# Autodesk Inventor assembly: 90 degree curved shooter v1
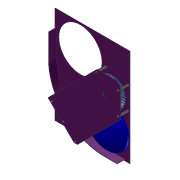
[picture p0: Inventor's stored thumbnail of the model, 180x180]
Saved by Autodesk Inventor 2012 (Build 160160000, 160)
## iProperties
Created: 2013-01-15
Part Number: 90 degree curved shooter v1
Document SubType Name: Assembly
Designer: William
Mass: 2029.94 g
Surface Area: 13536.5 cm^2
Volume: 1773.91 cm^3
Density: 1.14433 g/cm^3
Author: William
## Documents named in this file (10)
- Z:\UserData\Documents\Inventor\team1885frc\Robot2013\Launcher\90 degree curved shooter v1.iam
- Z:\UserData\Documents\Inventor\team1885frc\Robot2013\Launcher\Shooter Plate.ipt
- Z:\UserData\Documents\Inventor\team1885frc\Robot2013\Launcher\Shooter Curve.ipt
- Z:\UserData\Documents\Inventor\team1885frc\Hardware\Bearings\500id_1.125od_closed_flange_bearing.ipt
- Z:\UserData\Documents\Inventor\team1885frc\Robot2013\Game\disc.ipt
- Z:\UserData\Documents\Inventor\team1885frc\Robot2013\Launcher\Shooter Plate top.ipt
- Z:\UserData\Documents\Inventor\team1885frc\AndyMark\PneumaticWheel_am-0970\PneumaticWheel_am-0970.iam
- Z:\UserData\Documents\Inventor\team1885frc\VEXPro\VersaHub\217-2592.20121203.ipt
- Z:\UserData\Documents\Inventor\team1885frc\Robot2013\LauncherRearrange\UpperPlateStandoff.ipt
- Z:\UserData\Documents\Inventor\team1885frc\Hardware\Bolts\Bolt_0.25_20_0.75len_SocketHead.ipt
## Components (26 placed, 9 different names)
1. Shooter Plate:1 — Flush:1, Flush:2, Mate:3, Mate:16, Mate:100, Mate:101, Mate:121, Mate:122, Mate:123, Mate:124, Mate:125, Mate:126, Mate:136, Mate:137, Mate:138, Mate:139, Mate:140, Mate:141, Mate:151, Mate:152, Mate:153, Mate:163, Mate:164, Mate:165
2. Shooter Curve:1 — Flush:1, Flush:2, Mate:3, Tangent:1
3. disc:1 — Mate:16, Tangent:1
4. Shooter Plate top:1 — Mate:142, Mate:143, Mate:144, Mate:148, Mate:149, Mate:150, Mate:154, Mate:155, Mate:156, Mate:157, Mate:158, Mate:159
5. 500id_1.125od_closed_flange_bearing:7 — Mate:100, Mate:101, Mate:118, Mate:119
6. PneumaticWheel_am-0970:1 [sub-assembly] — Mate:113, Mate:114, Mate:115, Mate:116
7. 217-2592.20121203:1 — Mate:113, Mate:114, Mate:117, Mate:118
8. 217-2592.20121203:2 — Mate:115, Mate:116, Mate:117, Mate:119
9. UpperPlateStandoff:1 — Mate:121, Mate:126, Mate:142, Mate:143, Mate:145
10. UpperPlateStandoff:2 — Mate:122, Mate:125, Mate:144, Mate:147
11. UpperPlateStandoff:3 — Mate:123, Mate:124, Mate:146
12. Bolt_0.25_20_0.75len_SocketHead:1 — Mate:146, Mate:149
13. Bolt_0.25_20_0.75len_SocketHead:2 — Mate:147, Mate:150
14. Bolt_0.25_20_0.75len_SocketHead:3 — Mate:145, Mate:148
15. Bolt_0.25_20_0.75len_SocketHead:4 — Mate:140, Mate:141
16. Bolt_0.25_20_0.75len_SocketHead:5 — Mate:138, Mate:139
17. Bolt_0.25_20_0.75len_SocketHead:6 — Mate:136, Mate:137
18. Bolt_0.25_20_0.75len_SocketHead:7 — Mate:156, Mate:162
19. Bolt_0.25_20_0.75len_SocketHead:8 — Mate:165, Mate:167
20. Bolt_0.25_20_0.75len_SocketHead:9 — Mate:154, Mate:160
21. Bolt_0.25_20_0.75len_SocketHead:10 — Mate:155, Mate:161
22. Bolt_0.25_20_0.75len_SocketHead:11 — Mate:163, Mate:166
23. Bolt_0.25_20_0.75len_SocketHead:12 — Mate:164, Mate:168
24. UpperPlateStandoff:4 — Mate:151, Mate:157, Mate:160, Mate:166
25. UpperPlateStandoff:5 — Mate:152, Mate:158, Mate:161, Mate:167
26. UpperPlateStandoff:6 — Mate:153, Mate:159, Mate:162, Mate:168
## Relationships (53: Mate 50, Flush 2, Tangent 1)
- Flush:1 (-6.35 mm): Shooter Plate:1 ↔ Shooter Curve:1
- Flush:2 (6.35 mm): Shooter Plate:1 ↔ Shooter Curve:1
- Mate:3: Shooter Plate:1 ↔ Shooter Curve:1
- Mate:16: Shooter Plate:1 ↔ disc:1
- Mate:100: Shooter Plate:1 ↔ 500id_1.125od_closed_flange_bearing:7
- Mate:101: Shooter Plate:1 ↔ 500id_1.125od_closed_flange_bearing:7
- Tangent:1: Shooter Curve:1 ↔ disc:1
- Mate:113: PneumaticWheel_am-0970:1 ↔ 217-2592.20121203:1
- Mate:114: PneumaticWheel_am-0970:1 ↔ 217-2592.20121203:1
- Mate:115: PneumaticWheel_am-0970:1 ↔ 217-2592.20121203:2
- Mate:116: PneumaticWheel_am-0970:1 ↔ 217-2592.20121203:2
- Mate:117: 217-2592.20121203:1 ↔ 217-2592.20121203:2
- Mate:118 (3.175 mm): 500id_1.125od_closed_flange_bearing:7 ↔ 217-2592.20121203:1
- Mate:119: 500id_1.125od_closed_flange_bearing:7 ↔ 217-2592.20121203:2
- Mate:121: Shooter Plate:1 ↔ UpperPlateStandoff:1
- Mate:122: Shooter Plate:1 ↔ UpperPlateStandoff:2
- Mate:123: Shooter Plate:1 ↔ UpperPlateStandoff:3
- Mate:124: Shooter Plate:1 ↔ UpperPlateStandoff:3
- Mate:125: Shooter Plate:1 ↔ UpperPlateStandoff:2
- Mate:126: Shooter Plate:1 ↔ UpperPlateStandoff:1
- Mate:136: Shooter Plate:1 ↔ Bolt_0.25_20_0.75len_SocketHead:6
- Mate:137: Shooter Plate:1 ↔ Bolt_0.25_20_0.75len_SocketHead:6
- Mate:138: Shooter Plate:1 ↔ Bolt_0.25_20_0.75len_SocketHead:5
- Mate:139: Shooter Plate:1 ↔ Bolt_0.25_20_0.75len_SocketHead:5
- Mate:140: Shooter Plate:1 ↔ Bolt_0.25_20_0.75len_SocketHead:4
- Mate:141: Shooter Plate:1 ↔ Bolt_0.25_20_0.75len_SocketHead:4
- Mate:142: Shooter Plate top:1 ↔ UpperPlateStandoff:1
- Mate:143: Shooter Plate top:1 ↔ UpperPlateStandoff:1
- Mate:144: Shooter Plate top:1 ↔ UpperPlateStandoff:2
- Mate:145: UpperPlateStandoff:1 ↔ Bolt_0.25_20_0.75len_SocketHead:3
- Mate:146: UpperPlateStandoff:3 ↔ Bolt_0.25_20_0.75len_SocketHead:1
- Mate:147: UpperPlateStandoff:2 ↔ Bolt_0.25_20_0.75len_SocketHead:2
- Mate:148: Shooter Plate top:1 ↔ Bolt_0.25_20_0.75len_SocketHead:3
- Mate:149: Shooter Plate top:1 ↔ Bolt_0.25_20_0.75len_SocketHead:1
- Mate:150: Shooter Plate top:1 ↔ Bolt_0.25_20_0.75len_SocketHead:2
- Mate:151: Shooter Plate:1 ↔ UpperPlateStandoff:4
- Mate:152: Shooter Plate:1 ↔ UpperPlateStandoff:5
- Mate:153: Shooter Plate:1 ↔ UpperPlateStandoff:6
- Mate:154: Shooter Plate top:1 ↔ Bolt_0.25_20_0.75len_SocketHead:9
- Mate:155: Shooter Plate top:1 ↔ Bolt_0.25_20_0.75len_SocketHead:10
- Mate:156: Shooter Plate top:1 ↔ Bolt_0.25_20_0.75len_SocketHead:7
- Mate:157: Shooter Plate top:1 ↔ UpperPlateStandoff:4
- Mate:158: Shooter Plate top:1 ↔ UpperPlateStandoff:5
- Mate:159: Shooter Plate top:1 ↔ UpperPlateStandoff:6
- Mate:160: Bolt_0.25_20_0.75len_SocketHead:9 ↔ UpperPlateStandoff:4
- Mate:161: Bolt_0.25_20_0.75len_SocketHead:10 ↔ UpperPlateStandoff:5
- Mate:162: Bolt_0.25_20_0.75len_SocketHead:7 ↔ UpperPlateStandoff:6
- Mate:163: Shooter Plate:1 ↔ Bolt_0.25_20_0.75len_SocketHead:11
- Mate:164: Shooter Plate:1 ↔ Bolt_0.25_20_0.75len_SocketHead:12
- Mate:165: Shooter Plate:1 ↔ Bolt_0.25_20_0.75len_SocketHead:8
- Mate:166: Bolt_0.25_20_0.75len_SocketHead:11 ↔ UpperPlateStandoff:4
- Mate:167: Bolt_0.25_20_0.75len_SocketHead:8 ↔ UpperPlateStandoff:5
- Mate:168: Bolt_0.25_20_0.75len_SocketHead:12 ↔ UpperPlateStandoff:6
